# Autodesk Inventor assembly: Ball-Joint-Rod-Small
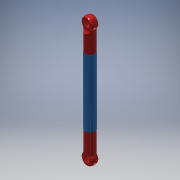
[picture p0: Inventor's stored thumbnail of the model, 180x180]
Saved by Autodesk Inventor 2018.2 (Build 222227000, 227)
## iProperties
Created: 2018-02-18
Part Number: Ball-Joint-Rod-Small
Material: Generisch
Document SubType Name: Assembly
Designer: JochenAlt
Author: JochenAlt
## Documents named in this file (4)
- D:\Projects\Donna\CAD\Ball-Joint-Rod-Small.iam
- D:\Projects\Donna\CAD\Ball-Joint Female.ipt
- D:\Projects\Donna\CAD\Ball-Joint-Rod-small.ipt
- D:\Projects\Donna\CAD\Stewart-Rod-Pipe-Small.ipt
## Components (4 placed, 3 different names)
1. Ball Joint Female:1 — Passend:3
2. Ball Joint Female:2 — Passend:1, Passend:2, Passend:5, Passend:6
3. Rod M2.5:1 — Passend:1, Passend:2, Passend:3, Passend:4
4. Stewart-Rod-Pipe-Small:1 — Passend:4, Passend:5
## Relationships (6: Mate 6)
- Passend:1 [Mate]: Ball Joint Female:2 ↔ Rod M2.5:1
- Passend:2 [Mate]: Ball Joint Female:2 ↔ Rod M2.5:1
- Passend:3 [Mate]: Ball Joint Female:1 ↔ Rod M2.5:1
- Passend:4 [Mate]: Rod M2.5:1 ↔ Stewart-Rod-Pipe-Small:1
- Passend:5 [Mate]: Ball Joint Female:2 ↔ Stewart-Rod-Pipe-Small:1
- Passend:6 [Mate]: Ball Joint Female:2
